# Autodesk Inventor assembly: lamp
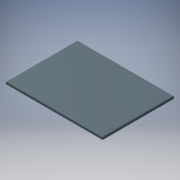
[picture p0: Inventor's stored thumbnail of the model, 180x180]
Saved by Autodesk Inventor 2016 (Build 200138000, 138)
## iProperties
Created: 2020-08-25
Part Number: lamp
Document SubType Name: Assembly
Designer: vtolenti89
Author: vtolenti89
## Documents named in this file (3)
- C:\Users\vtolenti89\Documents\05_Electronics\02-Projects\night-light-sensor\04-Mechanics\lamp.iam
- C:\Users\vtolenti89\Documents\05_Electronics\Kicad\Projects\Watering_System\mechanics\Main_PCB.ipt
- C:\Users\vtolenti89\Documents\05_Electronics\Kicad\Projects\Watering_System\mechanics\Solar_Panel.ipt
## Components (2 placed, 2 different names)
1. Main_PCB:1
2. Solar_Panel:1 — Flush:1
## Relationships (1: Flush 1)
- Flush:1: Solar_Panel:1
